# Autodesk Inventor assembly: Montagem integrada do eletroima
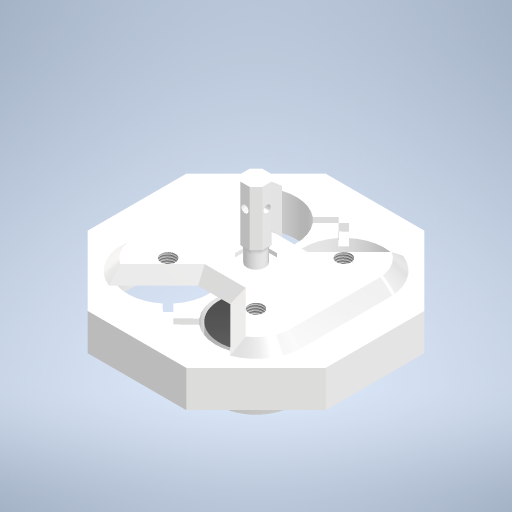
[picture p0: Inventor's stored thumbnail of the model, 512x512]
Saved by Autodesk Inventor 2023 (Build 270158000, 158)
## iProperties
Created: 2023-03-21
Part Number: Montagem integrada do eletroima
Document SubType Name: Assembly
Designer: Inteli
Author: Inteli
## Documents named in this file (3)
- C:\Users\Inteli\OneDrive\Modulos\Modulo 5\Eletroima\Montagem integrada do eletroima.iam
- C:\Users\Inteli\Documents\GitHub\grupo1\src\3d_models\Garra_Eletro_ima\Suporte_eletroima.ipt
- C:\Users\Inteli\Documents\GitHub\grupo1\src\3d_models\Garra_Eletro_ima\Eletroima.ipt
## Components (2 placed, 2 different names)
1. Suporte_eletroima:1 — Insert:1
2. Eletroima:1 — Insert:1
## Relationships (1: Insert 1)
- Insert:1: Suporte_eletroima:1 ↔ Eletroima:1
